# Autodesk Inventor assembly: differential gearbox compact
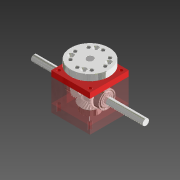
[picture p0: Inventor's stored thumbnail of the model, 180x180]
Saved by Autodesk Inventor 2020 (Build 240168000, 168)
## iProperties
Created: 2020-05-19
Part Number: differential gearbox compact
Document SubType Name: Assembly
Designer: stefa
Author: stefa
## Documents named in this file (11)
- D:\github_gedeeld\BeerMinder\3D-model\axis5_6\differential gearbox compact.iam
- D:\github_gedeeld\BeerMinder\3D-model\bearings\Ball Bearing 608ZZ.ipt
- D:\github_gedeeld\BeerMinder\3D-model\axis5_6\as bevelgear.ipt
- D:\github_gedeeld\BeerMinder\3D-model\axis5_6\tandwiel assemble.iam
- D:\github_gedeeld\BeerMinder\3D-model\axis5_6\gearbox v2.ipt
- D:\github_gedeeld\BeerMinder\3D-model\axis5_6\gearbox v2 mid part.ipt
- D:\github_gedeeld\BeerMinder\3D-model\axis5_6\as naar endeffector compact.ipt
- D:\github_gedeeld\BeerMinder\3D-model\axis5_6\endeffector mount as 8 compact.ipt
- D:\github_gedeeld\BeerMinder\3D-model\bearings\conische lager.ipt
- D:\github_gedeeld\BeerMinder\3D-model\axis5_6\conischLagerBlok.ipt
- D:\github_gedeeld\BeerMinder\3D-model\axis5_6\axis5_6 smaller v1\Design Accelerator\Bevel Gear11.ipt
## Components (13 placed, 10 different names)
1. Ball Bearing 608ZZ:1 — Mate:30, Flush:14, Mate:37
2. Ball Bearing 608ZZ:2 — Mate:18, Mate:29, Flush:13
3. Ball Bearing 608ZZ:3 — Mate:23, Flush:10, Mate:24, Flush:20
4. as bevelgear:2 — Mate:18, Mate:33, Mate:40, Mate:41, Flush:19
5. as naar endeffector compact:1 — Mate:22, Flush:9, Angle:1, Mate:34, Flush:20
6. endeffector mount as 8 compact:1 — Mate:22, Flush:9, Angle:1
7. tandwiel assemble:1 [sub-assembly] — Mate:24, Mate:34, Mate:38, Flush:18, Mate:39, Mate:42
8. gearbox v2:1 — Mate:23, Flush:10, Mate:26, Mate:27, Mate:28, Flush:11, Flush:12, Mate:31
9. gearbox v2 mid part:1 — Flush:11, Flush:12, Mate:29, Flush:13, Mate:30, Flush:14, Mate:31, Mate:33, Mate:35, Flush:15, Flush:16
10. conische lager:1 — Mate:36, Flush:17
11. conischLagerBlok:1 — Mate:35, Flush:15, Flush:16, Mate:36, Flush:17
12. as bevelgear:3 — Mate:37, Mate:38, Flush:18, Mate:39
13. Bevel Gear klein:1 — Mate:40, Mate:41, Flush:19, Mate:42
## Relationships (33: Mate 20, Flush 12, Angle 1)
- Mate:18: Ball Bearing 608ZZ:2 ↔ as bevelgear:2
- Mate:22: as naar endeffector compact:1 ↔ endeffector mount as 8 compact:1
- Flush:9: as naar endeffector compact:1 ↔ endeffector mount as 8 compact:1
- Angle:1 (0 deg): as naar endeffector compact:1 ↔ endeffector mount as 8 compact:1
- Mate:23: Ball Bearing 608ZZ:3 ↔ gearbox v2:1
- Flush:10: Ball Bearing 608ZZ:3 ↔ gearbox v2:1
- Mate:24: Ball Bearing 608ZZ:3 ↔ tandwiel assemble:1
- Mate:26: gearbox v2:1
- Mate:27: gearbox v2:1
- Mate:28: gearbox v2:1
- Flush:11: gearbox v2:1 ↔ gearbox v2 mid part:1
- Flush:12: gearbox v2:1 ↔ gearbox v2 mid part:1
- Mate:29: Ball Bearing 608ZZ:2 ↔ gearbox v2 mid part:1
- Flush:13: Ball Bearing 608ZZ:2 ↔ gearbox v2 mid part:1
- Mate:30: Ball Bearing 608ZZ:1 ↔ gearbox v2 mid part:1
- Flush:14: Ball Bearing 608ZZ:1 ↔ gearbox v2 mid part:1
- Mate:31: gearbox v2:1 ↔ gearbox v2 mid part:1
- Mate:33: as bevelgear:2 ↔ gearbox v2 mid part:1
- Mate:34: as naar endeffector compact:1 ↔ tandwiel assemble:1
- Mate:35: gearbox v2 mid part:1 ↔ conischLagerBlok:1
- Flush:15: gearbox v2 mid part:1 ↔ conischLagerBlok:1
- Flush:16: gearbox v2 mid part:1 ↔ conischLagerBlok:1
- Mate:36: conische lager:1 ↔ conischLagerBlok:1
- Flush:17: conische lager:1 ↔ conischLagerBlok:1
- Mate:37: Ball Bearing 608ZZ:1 ↔ as bevelgear:3
- Mate:38: tandwiel assemble:1 ↔ as bevelgear:3
- Flush:18: tandwiel assemble:1 ↔ as bevelgear:3
- Mate:39: tandwiel assemble:1 ↔ as bevelgear:3
- Mate:40: as bevelgear:2 ↔ Bevel Gear klein:1
- Mate:41: as bevelgear:2 ↔ Bevel Gear klein:1
- Flush:19: as bevelgear:2 ↔ Bevel Gear klein:1
- Mate:42 (6.962 mm): tandwiel assemble:1 ↔ Bevel Gear klein:1
- Flush:20 (-1 mm): Ball Bearing 608ZZ:3 ↔ as naar endeffector compact:1
